# Autodesk Inventor assembly: Triton2_asm
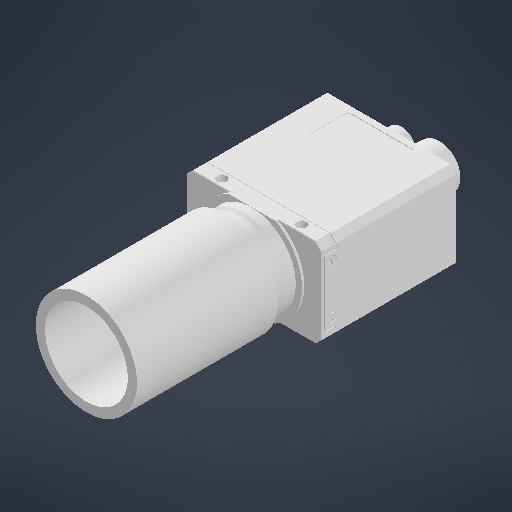
[picture p0: Inventor's stored thumbnail of the model, 512x512]
Saved by Autodesk Inventor 2026 (Build 300175000, 175)
## iProperties
Created: 2025-04-19
Part Number: Triton2_asm
Document SubType Name: Assembly
Designer: Charl
Author: Charl
## Documents named in this file (3)
- E:\School\Research\Inventor\Cover\Camera\Triton2_asm.iam
- E:\School\Research\Inventor\Cover\Camera\Triton2_Imported.ipt
- E:\School\Research\Inventor\Cover\Camera\LensTubing.ipt
## Components (2 placed, 2 different names)
1. Triton2_Imported:1 — Mate:1, Mate:2
2. LensTubing:1 — Mate:1, Mate:2
## Relationships (2: Mate 2)
- Mate:1: Triton2_Imported:1 ↔ LensTubing:1
- Mate:2: Triton2_Imported:1 ↔ LensTubing:1
